# Autodesk Inventor assembly: MagnetAssembly
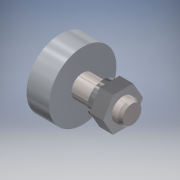
[picture p0: Inventor's stored thumbnail of the model, 180x180]
Saved by Autodesk Inventor 2017 (Build 210142000, 142)
## iProperties
Created: 2016-12-31
Part Number: MagnetAssembly
Document SubType Name: Assembly
Designer: umr
Author: umr
## Documents named in this file (4)
- D:\SeniorProject\Models2\UTM\MagnetAssembly.iam
- D:\SeniorProject\Models2\UTM\15mm x 5mm x 5mm Ring Magnet.ipt
- D:\SeniorProject\Models2\UTM\M5 Screw_16mm.ipt
- D:\SeniorProject\Models2\UTM\M5 Locknut.ipt
## Components (3 placed, 3 different names)
1. 15mm x 5mm x 5mm Ring Magnet:1 — Mate:22, Mate:23
2. M5 Screw_16mm:1 — Mate:22, Mate:23, Mate:24, Flush:2
3. M5 Locknut:1 — Mate:24, Flush:2
## Relationships (4: Mate 3, Flush 1)
- Mate:22: 15mm x 5mm x 5mm Ring Magnet:1 ↔ M5 Screw_16mm:1
- Mate:23: 15mm x 5mm x 5mm Ring Magnet:1 ↔ M5 Screw_16mm:1
- Mate:24: M5 Screw_16mm:1 ↔ M5 Locknut:1
- Flush:2 (2 mm): M5 Screw_16mm:1 ↔ M5 Locknut:1
